# Autodesk Inventor assembly: Tentacle Full
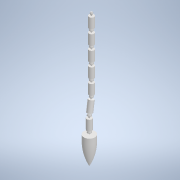
[picture p0: Inventor's stored thumbnail of the model, 180x180]
Saved by Autodesk Inventor 2022 (Build 260153000, 153)
## iProperties
Created: 2020-07-11
Part Number: Tentacle Full
Document SubType Name: Assembly
Designer: saipr
Author: saipr
## Documents named in this file (3)
- C:\Users\saipr\Desktop\Autodesk 2022\Builds\Parts\Tentacle Full.iam
- C:\Users\saipr\Desktop\Autodesk 2022\Builds\Parts\octopus tentacles.ipt
- C:\Users\saipr\Desktop\Autodesk 2022\Builds\Parts\octopus tentacle end.ipt
## Components (8 placed, 2 different names)
1. octopus tentacles:1 — Mate:1, Mate:2
2. octopus tentacles:2 — Mate:2, Mate:3
3. octopus tentacles:3 — Mate:3, Mate:4
4. octopus tentacles:4 — Mate:4, Mate:5
5. octopus tentacles:5 — Mate:5, Mate:6
6. octopus tentacles:6 — Mate:6, Mate:7
7. octopus tentacles:7 — Mate:7
8. octopus tentacle end:1 — Mate:1
## Relationships (7: Mate 7)
- Mate:1: octopus tentacles:1 ↔ octopus tentacle end:1
- Mate:2: octopus tentacles:1 ↔ octopus tentacles:2
- Mate:3: octopus tentacles:2 ↔ octopus tentacles:3
- Mate:4: octopus tentacles:3 ↔ octopus tentacles:4
- Mate:5: octopus tentacles:4 ↔ octopus tentacles:5
- Mate:6: octopus tentacles:5 ↔ octopus tentacles:6
- Mate:7: octopus tentacles:6 ↔ octopus tentacles:7
